# Autodesk Inventor assembly: Tractor_Plates
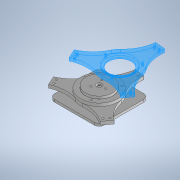
[picture p0: Inventor's stored thumbnail of the model, 180x180]
Saved by Autodesk Inventor 2022 (Build 260153070, 153G)
## iProperties
Created: 2022-03-05
Part Number: Tractor_Plates
Document SubType Name: Assembly
Designer: a laptop
Author: a laptop
## Documents named in this file (10)
- C:\Users\a laptop\Desktop\MDL_2021_Project\Tractor_Plates\Tractor_Plates.iam
- C:\Users\a laptop\Desktop\MDL_2021_Project\Tractor_Plates\Tractor_Static.ipt
- C:\Users\a laptop\Desktop\MDL_2021_Project\Tractor_Plates\Tractor_Mobile.ipt
- C:\Users\a laptop\Desktop\MDL_2021_Project\Tractor_Plates\Tractor_Plates\Design Accelerator\Bearing1.iam
- C:\Users\a laptop\Desktop\MDL_2021_Project\Tractor_Plates\Slip_Ring.ipt
- C:\Users\a laptop\Desktop\MDL_2021_Project\Tractor_Plates\Magnet.ipt
- C:\Users\a laptop\Desktop\MDL_2021_Project\Tractor_Plates\Tractor_Mobile_2.ipt
- C:\Users\a laptop\Desktop\MDL_2021_Project\Tractor_Plates\Tractor_Static_2.ipt
- C:\Users\a laptop\Desktop\MDL_2021_Project\Tractor_Plates\Tractor_Static_3.ipt
- C:\Users\a laptop\Desktop\MDL_2021_Project\Tractor_Plates\Tractor_Static_4.ipt
## Components (9 placed, 9 different names)
1. Bearing:1 [sub-assembly] — Mate:1, Mate:5, Mate:6, Mate:7
2. Slip_Ring:1 — Mate:2, Mate:15
3. Magnet:1 — Mate:3, Mate:16, Mate:17
4. Tractor_Static_4:1 — Mate:18, Mate:19, Mate:20
5. Tractor_Mobile:1 — Mate:6, Mate:7, Mate:8, Mate:9, Mate:10, Mate:11
6. Tractor_Mobile_2:1 — Mate:8, Mate:9, Mate:10, Mate:11
7. Tractor_Static_3:1
8. Tractor_Static_2:1 — Mate:12, Mate:13, Mate:14
9. Tractor_Static:1 — Mate:1, Mate:2, Mate:3, Mate:5, Mate:12, Mate:13, Mate:14, Mate:15, Mate:16, Mate:17, Mate:18, Mate:19, Mate:20
## Relationships (19: Mate 19)
- Mate:1: Bearing:1 ↔ Tractor_Static:1
- Mate:2: Slip_Ring:1 ↔ Tractor_Static:1
- Mate:3: Magnet:1 ↔ Tractor_Static:1
- Mate:5: Bearing:1 ↔ Tractor_Static:1
- Mate:6: Bearing:1 ↔ Tractor_Mobile:1
- Mate:7: Bearing:1 ↔ Tractor_Mobile:1
- Mate:8: Tractor_Mobile:1 ↔ Tractor_Mobile_2:1
- Mate:9: Tractor_Mobile:1 ↔ Tractor_Mobile_2:1
- Mate:10: Tractor_Mobile:1 ↔ Tractor_Mobile_2:1
- Mate:11: Tractor_Mobile:1 ↔ Tractor_Mobile_2:1
- Mate:12: Tractor_Static_2:1 ↔ Tractor_Static:1
- Mate:13: Tractor_Static_2:1 ↔ Tractor_Static:1
- Mate:14: Tractor_Static_2:1 ↔ Tractor_Static:1
- Mate:15: Slip_Ring:1 ↔ Tractor_Static:1
- Mate:16: Magnet:1 ↔ Tractor_Static:1
- Mate:17: Magnet:1 ↔ Tractor_Static:1
- Mate:18: Tractor_Static_4:1 ↔ Tractor_Static:1
- Mate:19: Tractor_Static_4:1 ↔ Tractor_Static:1
- Mate:20: Tractor_Static_4:1 ↔ Tractor_Static:1
